# Autodesk Inventor assembly: Gripper
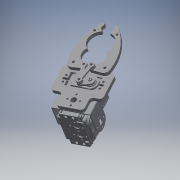
[picture p0: Inventor's stored thumbnail of the model, 180x180]
Saved by Autodesk Inventor 2016 (Build 200138000, 138)
## iProperties
Created: 2016-07-07
Part Number: Gripper
Document SubType Name: Assembly
Designer: lachesis
Author: lachesis
## Documents named in this file (9)
- C:\Users\lachesis\git\Swarmie-Build\Swarmie-Assembly\Assemblies\Gripper.iam
- C:\Users\lachesis\git\Swarmie-Build\Swarmie-Assembly\Parts\GripperServoBracket.ipt
- C:\Users\lachesis\git\Swarmie-Build\Swarmie-Assembly\Parts\GripperServo\Servo.iam
- C:\Users\lachesis\git\Swarmie-Build\Swarmie-Assembly\Parts\GripperCBracket.ipt
- C:\Users\lachesis\git\Swarmie-Build\Swarmie-Assembly\Parts\GripperWristPlate.ipt
- C:\Users\lachesis\git\Swarmie-Build\Swarmie-Assembly\Parts\GripperFinger.ipt
- C:\Users\lachesis\git\Swarmie-Build\Swarmie-Assembly\Parts\GripperServoArm.ipt
- C:\Users\lachesis\git\Swarmie-Build\Swarmie-Assembly\Parts\GripperSpacer.ipt
- C:\Users\lachesis\git\Swarmie-Build\Swarmie-Assembly\Parts\GripperServoHorn.ipt
## Components (11 placed, 8 different names)
1. GripperServoBracket:1 — Mate:5, Mate:14, Mate:15, Mate:16, Mate:18
2. Servo:1 [sub-assembly] — Mate:14, Mate:15, Mate:16, Mate:17
3. GripperCBracket:1 — Mate:5, Mate:8, Mate:17, Mate:18, Mate:19, Mate:20
4. GripperWristPlate:1 — Mate:8, Mate:11, Mate:19, Mate:20, Mate:21, Mate:22, Rotational:1, Rotational:2
5. Servo:2 [sub-assembly] — Mate:11, Mate:21, Mate:22, Mate:26
6. GripperFinger:1 — Rotational:1, Mate:24, Mate:25
7. GripperFinger:2 — Rotational:2, Rotational:5
8. GripperServoArm:2 — Rotational:6, Mate:29
9. GripperServoArm:3 — Rotational:5, Mate:27, Mate:28, Mate:29
10. GripperSpacer:1 — Mate:24, Mate:25, Rotational:6
11. GripperServoHorn:1 — Mate:26, Mate:27, Mate:28
## Relationships (22: Mate 18, RevoluteJoint 4)
- Mate:5: GripperServoBracket:1 ↔ GripperCBracket:1
- Mate:8: GripperCBracket:1 ↔ GripperWristPlate:1
- Mate:11: GripperWristPlate:1 ↔ Servo:2
- Mate:14: GripperServoBracket:1 ↔ Servo:1
- Mate:15: GripperServoBracket:1 ↔ Servo:1
- Mate:16: GripperServoBracket:1 ↔ Servo:1
- Mate:17: Servo:1 ↔ GripperCBracket:1
- Mate:18: GripperServoBracket:1 ↔ GripperCBracket:1
- Mate:19: GripperCBracket:1 ↔ GripperWristPlate:1
- Mate:20: GripperCBracket:1 ↔ GripperWristPlate:1
- Mate:21: GripperWristPlate:1 ↔ Servo:2
- Mate:22 (0.254 mm): GripperWristPlate:1 ↔ Servo:2
- Rotational:1 [RevoluteJoint]: GripperWristPlate:1 ↔ GripperFinger:1
- Rotational:2 [RevoluteJoint]: GripperWristPlate:1 ↔ GripperFinger:2
- Rotational:5 [RevoluteJoint]: GripperFinger:2 ↔ GripperServoArm:3
- Mate:24: GripperFinger:1 ↔ GripperSpacer:1
- Mate:25: GripperFinger:1 ↔ GripperSpacer:1
- Rotational:6 [RevoluteJoint]: GripperServoArm:2 ↔ GripperSpacer:1
- Mate:26: Servo:2 ↔ GripperServoHorn:1
- Mate:27: GripperServoArm:3 ↔ GripperServoHorn:1
- Mate:28: GripperServoArm:3 ↔ GripperServoHorn:1
- Mate:29: GripperServoArm:2 ↔ GripperServoArm:3
